# Autodesk Inventor assembly: VP MCMASTER 1569A978 AI 
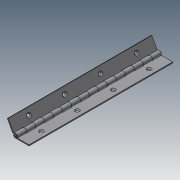
[picture p0: Inventor's stored thumbnail of the model, 180x180]
Saved by Autodesk Inventor 2018.3 (Build 223284000, 284)
## iProperties
Created: 2019-10-29
Vendor: HHMI: JRC - ID&F
Document SubType Name: Assembly
Designer: arnoldj
RuleStatus: InUse
AfterDocSave0: file://Part Number Cleaner
DESIGN DEPARTMENT: HHMI: JRC - ID&F
ALTERED ITEM PART NUMBER: N/A
ALTERED ITEM VENDOR: N/A
ALTERED ITEM DESCRIPTION: N/A
Author: arnoldj
Revision Number: 0
## Documents named in this file (3)
- C:\_WORKSPACE\DATA\PROJECTS\_PROJECTS BY LAB\FLY FACILITY\FLY MEDIA VIAL PLUGGING\VP MCMASTER 1569A978 AI .iam
- C:\_WORKSPACE\DATA\PROJECTS\_PROJECTS BY LAB\FLY FACILITY\FLY MEDIA VIAL PLUGGING\VP MCMASTER 1569A978 AI_A .ipt
- C:\_WORKSPACE\DATA\PROJECTS\_PROJECTS BY LAB\FLY FACILITY\FLY MEDIA VIAL PLUGGING\VP MCMASTER 1569A978 AI_B .ipt
## Components (2 placed, 2 different names)
1. VP MCMASTER 1569A978 AI_A :1 — Flush:1, Mate:1
2. VP MCMASTER 1569A978 AI_B :1 — Flush:1, Mate:1
## Relationships (2: Flush 1, Mate 1)
- Flush:1: VP MCMASTER 1569A978 AI_A :1 ↔ VP MCMASTER 1569A978 AI_B :1
- Mate:1: VP MCMASTER 1569A978 AI_A :1 ↔ VP MCMASTER 1569A978 AI_B :1
